# Autodesk Inventor assembly: Light Saber Inventor Native
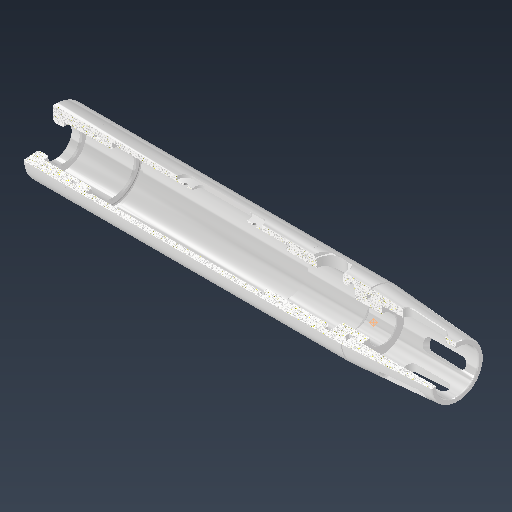
[picture p0: Inventor's stored thumbnail of the model, 512x512]
Saved by Autodesk Inventor 2025.1 (Build 291241000, 241)
## iProperties
Manager: Michael A. Lacey
Company: Personal
Created: 2024-08-20
Part Number: Light Saber Inventor Native
Document SubType Name: Assembly
Designer: Michael A. Lacey
Project: Light Saber
Description: Inventor Recreation
Engineer: Michael A. Lacey
Mass: 307.395 g
Surface Area: 616.009 cm^2
Volume: 113.85 cm^3
Author: Michael A. Lacey
Title: LightSaber
Subject: PropBody
## Documents named in this file (5)
- E:\Michael\Documents\GitHub Repos\LightSaber\CAD Files\Rev 3 - Most recent (i think)\Inventor\inventorNative.iam
- E:\Michael\Documents\GitHub Repos\LightSaber\CAD Files\Rev 3 - Most recent (i think)\Inventor\InventorNativeCentralControl.ipt
- E:\Michael\Documents\GitHub Repos\LightSaber\CAD Files\Rev 3 - Most recent (i think)\Inventor\InventorNativeEmitter.ipt
- E:\Michael\Documents\GitHub Repos\LightSaber\CAD Files\Rev 3 - Most recent (i think)\Inventor\InventorNativeNewHilt.ipt
- E:\Michael\Documents\GitHub Repos\LightSaber\CAD Files\Rev 3 - Most recent (i think)\Inventor\PommelPart.ipt
## Components (4 placed, 4 different names)
1. InventorNativeCentralControl:1 — Mate:1, Mate:3, Mate:4, Mate:5
2. InventorNativeEmitter:1 — Mate:2, Mate:3, Mate:5, Mate:6
3. InventorNativeNewHilt:1 — Mate:1, Mate:2, Mate:4, Mate:6, Mate:7, Mate:8, Mate:9
4. PommelPart:1 — Mate:7, Mate:8, Mate:9
## Relationships (9: Mate 9)
- Mate:1: InventorNativeCentralControl:1 ↔ InventorNativeNewHilt:1
- Mate:2: InventorNativeEmitter:1 ↔ InventorNativeNewHilt:1
- Mate:3: InventorNativeCentralControl:1 ↔ InventorNativeEmitter:1
- Mate:4: InventorNativeCentralControl:1 ↔ InventorNativeNewHilt:1
- Mate:5: InventorNativeCentralControl:1 ↔ InventorNativeEmitter:1
- Mate:6: InventorNativeEmitter:1 ↔ InventorNativeNewHilt:1
- Mate:7: InventorNativeNewHilt:1 ↔ PommelPart:1
- Mate:8: InventorNativeNewHilt:1 ↔ PommelPart:1
- Mate:9: InventorNativeNewHilt:1 ↔ PommelPart:1
## Named parameters: Finish1_Area = 517.734, Finish2_Area = 517.734, Finish3_Area = 603.294
note: some values were not read from the file. Shown as the stored number, unit unknown: "Finish1_Area", "Finish2_Area", "Finish3_Area".
